# Autodesk Inventor assembly: Сборка_Конечная
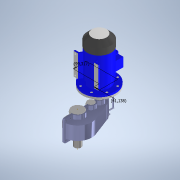
[picture p0: Inventor's stored thumbnail of the model, 180x180]
Saved by Autodesk Inventor 2021 (Build 250183000, 183)
## iProperties
Created: 2023-04-17
Part Number: Сборка_Конечная
Document SubType Name: Assembly
Designer: gdevc
Mass: 20589.9 g
Surface Area: 13395.2 cm^2
Volume: 12295.4 cm^3
Density: 1.6746 g/cm^3
Author: gdevc
## Documents named in this file (17)
- C:\Users\gdevc\OneDrive\Рабочий стол\Курсач\DetaliMashine\Новая папка\Сборка_Конечная.iam
- C:\Users\gdevc\OneDrive\Рабочий стол\Курсач\DetaliMashine\Новая папка\Корпус.v.2.0.iam
- C:\Users\gdevc\OneDrive\Рабочий стол\Курсач\DetaliMashine\Новая папка\Вал_тихоходный.ipt
- C:\Users\gdevc\OneDrive\Рабочий стол\Курсач\DetaliMashine\Новая папка\Вал_промежуточный.ipt
- C:\Users\gdevc\OneDrive\Рабочий стол\Курсач\DetaliMashine\Новая папка\Валл быстроходный.ipt
- C:\Users\gdevc\OneDrive\Рабочий стол\Курсач\DetaliMashine\Новая папка\Крышка, тихая.ipt
- C:\Users\gdevc\OneDrive\Рабочий стол\Курсач\DetaliMashine\Новая папка\Крышка тих_выход.ipt
- C:\Users\gdevc\OneDrive\Рабочий стол\Курсач\DetaliMashine\Новая папка\Подшипник 205 ГОСТ 8338-75.ipt
- C:\Users\gdevc\OneDrive\Рабочий стол\Курсач\DetaliMashine\Новая папка\Крышка_пром.ipt
- C:\Users\gdevc\OneDrive\Рабочий стол\Курсач\DetaliMashine\Новая папка\Подшипник 210 ГОСТ 8338-75.ipt
- C:\Users\gdevc\OneDrive\Рабочий стол\Курсач\DetaliMashine\Новая папка\Колесо быстроходное.ipt
- C:\Users\gdevc\OneDrive\Рабочий стол\Курсач\DetaliMashine\Новая папка\Манжет 2-50x65x8 ГОСТ 8752-79.ipt
- C:\Users\gdevc\OneDrive\Рабочий стол\Курсач\DetaliMashine\Новая папка\Манжет 1-30x47x7 ГОСТ 8752-79.ipt
- C:\Users\gdevc\OneDrive\Рабочий стол\Курсач\DetaliMashine\Новая папка\Крышка_быстроходного.ipt
- C:\Users\gdevc\OneDrive\Рабочий стол\Курсач\DetaliMashine\Новая папка\Промежуточное колесо резина.ipt
- C:\Users\gdevc\OneDrive\Рабочий стол\Курсач\DetaliMashine\Новая папка\Резина конец.ipt
- C:\Users\gdevc\Downloads\Telegram Desktop\АИР100L IM2081 (2,4,6,8 пол)....ipt
## Components (19 placed, 16 different names)
1. Корпус.v.2.0:1 [sub-assembly] — Совмещение:3, Совмещение:4, Совмещение:6, Совмещение:7, Совмещение:8, Совмещение:11, Совмещение:12, Совмещение:14, Совмещение:15, Совмещение:16, Совмещение:17, Совмещение:18, Совмещение:19, Совмещение:20, Совмещение:21, Совмещение:29, Заподлицо:3, Совмещение:32
2. Вал_тихоходный:1 — Совмещение:1, Совмещение:5, Совмещение:22, Совмещение:25, Совмещение:31
3. Вал_промежуточный:1 — Совмещение:4, Совмещение:9, Совмещение:10, Совмещение:13, Совмещение:23, Совмещение:24
4. Валл быстроходный:1 — Совмещение:3, Заподлицо:1, Угол:1, Совмещение:27, Совмещение:28, Совмещение:33
5. Крышка, тихая:1 — Совмещение:5, Совмещение:6
6. Крышка тих_выход:1 — Совмещение:7, Совмещение:8, Совмещение:26
7. Подшипник 205 ГОСТ 8338-75:1 — Совмещение:9, Совмещение:10, Совмещение:11, Угол:3
8. Подшипник 205 ГОСТ 8338-75:2 — Совмещение:12, Совмещение:13, Угол:2
9. Крышка_пром:1 — Совмещение:15, Совмещение:17
10. Крышка_пром:2 — Совмещение:14, Совмещение:16
11. Подшипник 210 ГОСТ 8338-75:1 — Совмещение:18, Совмещение:19
12. Подшипник 210 ГОСТ 8338-75:2 — Совмещение:20, Совмещение:21, Совмещение:22
13. Колесо быстроходное:1 — Совмещение:23, Совмещение:24, Заподлицо:1, Заподлицо:2
14. Манжет 2-50x65x8 ГОСТ 8752-79:1 — Совмещение:25, Совмещение:26
15. Манжет 1-30x47x7 ГОСТ 8752-79:1 — Совмещение:27, Совмещение:30
16. Крышка_быстроходного:1 — Совмещение:28, Совмещение:29, Совмещение:30, Совмещение:34, Угол:5
17. Промежуточное колесо резина:1 — Совмещение:31, Заподлицо:2
18. Резина конец:1 — Заподлицо:3, Совмещение:32
19. АИР100L IM2081 (2,4,6,8 пол)...:1 — Совмещение:33, Угол:4, Совмещение:34
## Relationships (41: Mate 33, Angle 5, Flush 3)
- Совмещение:1 [Mate]: Вал_тихоходный:1
- Совмещение:3 [Mate]: Корпус.v.2.0:1 ↔ Валл быстроходный:1
- Совмещение:4 [Mate]: Корпус.v.2.0:1 ↔ Вал_промежуточный:1
- Совмещение:5 [Mate]: Вал_тихоходный:1 ↔ Крышка, тихая:1
- Совмещение:6 [Mate]: Корпус.v.2.0:1 ↔ Крышка, тихая:1
- Совмещение:7 [Mate]: Корпус.v.2.0:1 ↔ Крышка тих_выход:1
- Совмещение:8 [Mate]: Корпус.v.2.0:1 ↔ Крышка тих_выход:1
- Совмещение:9 [Mate]: Вал_промежуточный:1 ↔ Подшипник 205 ГОСТ 8338-75:1
- Совмещение:10 [Mate]: Вал_промежуточный:1 ↔ Подшипник 205 ГОСТ 8338-75:1
- Совмещение:11 [Mate]: Корпус.v.2.0:1 ↔ Подшипник 205 ГОСТ 8338-75:1
- Совмещение:12 [Mate]: Корпус.v.2.0:1 ↔ Подшипник 205 ГОСТ 8338-75:2
- Совмещение:13 [Mate]: Вал_промежуточный:1 ↔ Подшипник 205 ГОСТ 8338-75:2
- Совмещение:14 [Mate]: Корпус.v.2.0:1 ↔ Крышка_пром:2
- Совмещение:15 [Mate]: Корпус.v.2.0:1 ↔ Крышка_пром:1
- Совмещение:16 [Mate]: Корпус.v.2.0:1 ↔ Крышка_пром:2
- Совмещение:17 [Mate]: Корпус.v.2.0:1 ↔ Крышка_пром:1
- Совмещение:18 [Mate]: Корпус.v.2.0:1 ↔ Подшипник 210 ГОСТ 8338-75:1
- Совмещение:19 [Mate]: Корпус.v.2.0:1 ↔ Подшипник 210 ГОСТ 8338-75:1
- Совмещение:20 [Mate]: Корпус.v.2.0:1 ↔ Подшипник 210 ГОСТ 8338-75:2
- Совмещение:21 [Mate]: Корпус.v.2.0:1 ↔ Подшипник 210 ГОСТ 8338-75:2
- Совмещение:22 [Mate]: Вал_тихоходный:1 ↔ Подшипник 210 ГОСТ 8338-75:2
- Совмещение:23 [Mate]: Вал_промежуточный:1 ↔ Колесо быстроходное:1
- Совмещение:24 [Mate]: Вал_промежуточный:1 ↔ Колесо быстроходное:1
- Заподлицо:1 [Flush] (-1 mm): Валл быстроходный:1 ↔ Колесо быстроходное:1
- Угол:1 [Angle] (0 deg): Валл быстроходный:1
- Угол:2 [Angle] (90 deg): Подшипник 205 ГОСТ 8338-75:2
- Угол:3 [Angle] (90 deg): Подшипник 205 ГОСТ 8338-75:1
- Совмещение:25 [Mate]: Вал_тихоходный:1 ↔ Манжет 2-50x65x8 ГОСТ 8752-79:1
- Совмещение:26 [Mate]: Крышка тих_выход:1 ↔ Манжет 2-50x65x8 ГОСТ 8752-79:1
- Совмещение:27 [Mate]: Валл быстроходный:1 ↔ Манжет 1-30x47x7 ГОСТ 8752-79:1
- Совмещение:28 [Mate]: Валл быстроходный:1 ↔ Крышка_быстроходного:1
- Совмещение:29 [Mate]: Корпус.v.2.0:1 ↔ Крышка_быстроходного:1
- Совмещение:30 [Mate]: Манжет 1-30x47x7 ГОСТ 8752-79:1 ↔ Крышка_быстроходного:1
- Совмещение:31 [Mate]: Вал_тихоходный:1 ↔ Промежуточное колесо резина:1
- Заподлицо:2 [Flush] (-1 mm): Колесо быстроходное:1 ↔ Промежуточное колесо резина:1
- Заподлицо:3 [Flush]: Корпус.v.2.0:1 ↔ Резина конец:1
- Совмещение:32 [Mate]: Корпус.v.2.0:1 ↔ Резина конец:1
- Совмещение:33 [Mate]: Валл быстроходный:1 ↔ АИР100L IM2081 (2,4,6,8 пол)...:1
- Угол:4 [Angle] (0 deg): АИР100L IM2081 (2,4,6,8 пол)...:1
- Совмещение:34 [Mate]: Крышка_быстроходного:1 ↔ АИР100L IM2081 (2,4,6,8 пол)...:1
- Угол:5 [Angle] (0 deg): Крышка_быстроходного:1
